# Autodesk Inventor assembly: new_assembly
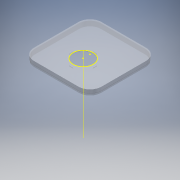
[picture p0: Inventor's stored thumbnail of the model, 180x180]
Saved by Autodesk Inventor 2019 (Build 230136000, 136)
## iProperties
Created: 2019-01-15
Part Number: new_assembly
Document SubType Name: Assembly
Designer: assman
Author: assman
## Documents named in this file (6)
- D:\Inventor\Projects\CatFeeder\version3 (new assembly)\new_assembly.iam
- D:\Inventor\Projects\CatFeeder\Case\version2\case_bottom.ipt
- D:\Inventor\Projects\CatFeeder\Case\version2\case_top.ipt
- D:\Inventor\Projects\CatFeeder\Jar\Jar.ipt
- D:\Inventor\Projects\CatFeeder\JarCone\version2\cono_nuevo.ipt
- D:\Inventor\Projects\CatFeeder\JarCone\version2\adaptador_cono.ipt
## Components (5 placed, 5 different names)
1. case_top:1 — Rigid:1, Rigid:4
2. case_bottom:1 — Rigid:1
3. Jar:1 — Rigid:2
4. cono_nuevo:1 — Rigid:2, Rigid:3
5. adaptador_cono:1 — Rigid:3, Rigid:4
## Relationships (4: WeldJoint 4)
- Rigid:1 [WeldJoint]: case_top:1 ↔ case_bottom:1
- Rigid:2 [WeldJoint]: Jar:1 ↔ cono_nuevo:1
- Rigid:3 [WeldJoint]: cono_nuevo:1 ↔ adaptador_cono:1
- Rigid:4 [WeldJoint]: case_top:1 ↔ adaptador_cono:1
